# Autodesk Inventor assembly: Assembly3
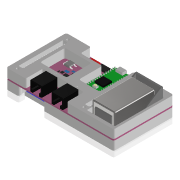
[picture p0: Inventor's stored thumbnail of the model, 180x180]
Saved by Autodesk Inventor 2020 (Build 240168000, 168)
## iProperties
Created: 2021-07-01
Part Number: Assembly3
Document SubType Name: Assembly
Designer: ferrerx
Author: ferrerx
## Documents named in this file (11)
- C:\Users\ferrerx\Desktop\Sport analyzer\Sport Analyzer 1.0.1\Mechanical\Assembly3.iam
- C:\Users\ferrerx\Desktop\Sport analyzer\Sport Analyzer 1.0.1\Mechanical\Sport Analyzer 1.0.1 PCB .iam
- C:\Users\ferrerx\Desktop\Sport analyzer\Sport Analyzer 1.0.1\Mechanical\Bottom PMMA.ipt
- C:\Users\ferrerx\Desktop\Sport analyzer\Sport Analyzer 1.0.1\Mechanical\Middle PMMA.ipt
- C:\Users\ferrerx\Desktop\Sport analyzer\Sport Analyzer 1.0.1\Mechanical\Top PMMA.ipt
- C:\Users\ferrerx\Desktop\Sport analyzer\Sport Analyzer 1.0.1\Mechanical\Adafruit 2.8TFT.ipt
- C:\Users\ferrerx\Desktop\Sport analyzer\Sport Analyzer 1.0.1\Mechanical\RJ12 Connector.ipt
- C:\Users\ferrerx\Desktop\Sport analyzer\Sport Analyzer 1.0.1\Mechanical\9V Battery.ipt
- C:\Users\ferrerx\Desktop\Sport analyzer\Sport Analyzer 1.0.1\Mechanical\Body_Housing 9V Battery.ipt
- C:\Users\ferrerx\Desktop\Sport analyzer\Sport Analyzer 1.0.1\Mechanical\Teensy3.2.ipt
- C:\Users\ferrerx\Desktop\Sport analyzer\Sport Analyzer 1.0.1\Mechanical\Sport Analyzer 1.0.1 PCB (2) .ipt
## Components (11 placed, 10 different names)
1. Sport Analyzer 1.0.1 PCB :1 [sub-assembly] — Mate:1, Flush:1, Flush:2, Mate:2, Flush:7, Mate:3, Mate:4, Mate:10, Mate:11, Mate:12, Mate:15, Mate:16, Mate:17, Flush:9, Flush:10, Mate:18
2. Bottom PMMA:1 — Mate:1, Flush:1, Flush:2, Flush:3, Flush:4, Flush:8
3. Middle PMMA:1 — Flush:3, Mate:2, Flush:4, Flush:5, Flush:6, Mate:5, Angle:1, Mate:13
4. Top PMMA:1 — Flush:5, Flush:6, Mate:14
5. Adafruit 2.8TFT:1 — Mate:5, Angle:1, Mate:13, Mate:14
6. RJ12 Connector:1 — Flush:7, Mate:3
7. RJ12 Connector:2 — Mate:4, Flush:8
8. 9V Battery:1 — Mate:7, Mate:8, Mate:9
9. Body_Housing 9V Battery:1 — Mate:7, Mate:8, Mate:9, Mate:10, Mate:11, Mate:12
10. Teensy3.2:1 — Mate:15, Mate:16, Mate:17
11. Sport Analyzer 1.0.1 PCB (2) :1 — Flush:9, Flush:10, Mate:18
## Relationships (28: Mate 17, Flush 10, Angle 1)
- Mate:1: Sport Analyzer 1.0.1 PCB :1 ↔ Bottom PMMA:1
- Flush:1: Sport Analyzer 1.0.1 PCB :1 ↔ Bottom PMMA:1
- Flush:2: Sport Analyzer 1.0.1 PCB :1 ↔ Bottom PMMA:1
- Flush:3: Bottom PMMA:1 ↔ Middle PMMA:1
- Mate:2: Sport Analyzer 1.0.1 PCB :1 ↔ Middle PMMA:1
- Flush:4: Bottom PMMA:1 ↔ Middle PMMA:1
- Flush:5: Middle PMMA:1 ↔ Top PMMA:1
- Flush:6: Middle PMMA:1 ↔ Top PMMA:1
- Flush:7: Sport Analyzer 1.0.1 PCB :1 ↔ RJ12 Connector:1
- Mate:3: Sport Analyzer 1.0.1 PCB :1 ↔ RJ12 Connector:1
- Mate:4: Sport Analyzer 1.0.1 PCB :1 ↔ RJ12 Connector:2
- Flush:8: Bottom PMMA:1 ↔ RJ12 Connector:2
- Mate:5: Middle PMMA:1 ↔ Adafruit 2.8TFT:1
- Angle:1 (0 deg): Middle PMMA:1 ↔ Adafruit 2.8TFT:1
- Mate:7: 9V Battery:1 ↔ Body_Housing 9V Battery:1
- Mate:8: 9V Battery:1 ↔ Body_Housing 9V Battery:1
- Mate:9 (1 mm): 9V Battery:1 ↔ Body_Housing 9V Battery:1
- Mate:10: Sport Analyzer 1.0.1 PCB :1 ↔ Body_Housing 9V Battery:1
- Mate:11: Sport Analyzer 1.0.1 PCB :1 ↔ Body_Housing 9V Battery:1
- Mate:12: Sport Analyzer 1.0.1 PCB :1 ↔ Body_Housing 9V Battery:1
- Mate:13: Middle PMMA:1 ↔ Adafruit 2.8TFT:1
- Mate:14: Top PMMA:1 ↔ Adafruit 2.8TFT:1
- Mate:15: Sport Analyzer 1.0.1 PCB :1 ↔ Teensy3.2:1
- Mate:16: Sport Analyzer 1.0.1 PCB :1 ↔ Teensy3.2:1
- Mate:17: Sport Analyzer 1.0.1 PCB :1 ↔ Teensy3.2:1
- Flush:9: Sport Analyzer 1.0.1 PCB :1 ↔ Sport Analyzer 1.0.1 PCB (2) :1
- Flush:10: Sport Analyzer 1.0.1 PCB :1 ↔ Sport Analyzer 1.0.1 PCB (2) :1
- Mate:18: Sport Analyzer 1.0.1 PCB :1 ↔ Sport Analyzer 1.0.1 PCB (2) :1
